# Autodesk Inventor assembly: Omni_Section
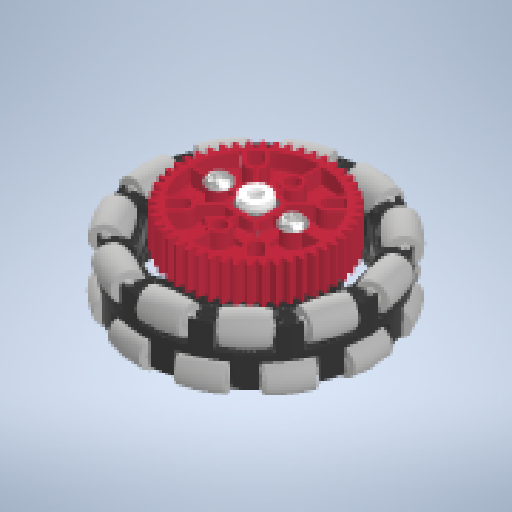
[picture p0: Inventor's stored thumbnail of the model, 512x512]
Saved by Autodesk Inventor 2025.2 (Build 292293000, 293)
## iProperties
Created: 2024-12-08
Part Number: Omni_Section
Document SubType Name: Assembly
Designer: Aditya Koduri
Author: Aditya Koduri
## Documents named in this file (13)
- C:\Users\joshi\Desktop\3388K CAD\Omni_Section.iam
- C:\Users\joshi\Desktop\3388K CAD\VEX Main\Structure\Hardware\Screw Steel - Hex\SScrew Hex Smooth 1.250.ipt
- C:\Users\joshi\Desktop\3388K CAD\VEX Main\Motion\Gears\HS Gear\HS 48T Gear, No Insert.iam
- C:\Users\joshi\Desktop\3388K CAD\VEX Main\Structure\Hardware\Nut Thin Nylock.ipt
- C:\Users\joshi\Desktop\3388K CAD\VEX Main\Motion\Wheels\Omni Wheel\3.25 Omni, No Insert.iam
- C:\Users\joshi\Desktop\3388K CAD\VEX Main\Motion\Insert Circle.ipt
- C:\Users\joshi\Desktop\3388K CAD\VEX Main\Motion\Spacers\Washer Teflon\TWasher .375 OD x .03125.ipt
- C:\Users\joshi\Desktop\3388K CAD\VEX Main\Motion\Spacers\Spacer Nylon .313 OD\NSpacer .313 OD x .250.ipt
- C:\Users\mzart\Downloads\VEX-CAD-Inventor-main\VEX-CAD-Inventor-main\Structure\Hardware\Screw Steel - Hex.ipt
- C:\Users\mzart\Downloads\VEX-CAD-Inventor-main\VEX-CAD-Inventor-main\Motion\Gears\HS Gear.iam
- C:\Users\mzart\Downloads\VEX-CAD-Inventor-main\VEX-CAD-Inventor-main\Motion\Wheels\Omni Wheel.iam
- C:\Users\mzart\Downloads\VEX-CAD-Inventor-main\VEX-CAD-Inventor-main\Motion\Spacers\Washer Teflon.ipt
- C:\Users\mzart\Downloads\VEX-CAD-Inventor-main\VEX-CAD-Inventor-main\Motion\Spacers\Spacer Nylon .313 OD.ipt
## Components (13 placed, 7 different names)
1. SScrew Hex Smooth 1.250:1
2. HS 48T Gear, No Insert:1 [sub-assembly] — Insert:10
3. Nut Thin Nylock:1
4. 3.25 Omni, No Insert:1 [sub-assembly] — Insert:11
5. SScrew Hex Smooth 1.250:2
6. Nut Thin Nylock:2
7. Insert Circle:1 — Insert:10, Insert:17
8. Insert Circle:2 — Insert:11, Insert:20
9. TWasher .375 OD x .03125:1 — Insert:18
10. TWasher .375 OD x .03125:2 — Insert:17, Insert:18
11. NSpacer .313 OD x .250:2 — Insert:19, Insert:20
12. TWasher .375 OD x .03125:3 — Insert:19, Insert:21
13. TWasher .375 OD x .03125:4 — Insert:21
## Relationships (13: Insert 13)
- [Insert]: HS 48T Gear, No Insert:1 ↔ 3.25 Omni, No Insert:1
- [Insert]: HS 48T Gear, No Insert:1 ↔ 3.25 Omni, No Insert:1
- [Insert]: SScrew Hex Smooth 1.250:1 ↔ HS 48T Gear, No Insert:1
- [Insert]: HS 48T Gear, No Insert:1 ↔ SScrew Hex Smooth 1.250:2
- [Insert]: Nut Thin Nylock:1 ↔ 3.25 Omni, No Insert:1
- [Insert]: 3.25 Omni, No Insert:1 ↔ Nut Thin Nylock:2
- Insert:10: HS 48T Gear, No Insert:1 ↔ Insert Circle:1
- Insert:11: 3.25 Omni, No Insert:1 ↔ Insert Circle:2
- Insert:17: Insert Circle:1 ↔ TWasher .375 OD x .03125:2
- Insert:18: TWasher .375 OD x .03125:1 ↔ TWasher .375 OD x .03125:2
- Insert:19: NSpacer .313 OD x .250:2 ↔ TWasher .375 OD x .03125:3
- Insert:20: Insert Circle:2 ↔ NSpacer .313 OD x .250:2
- Insert:21: TWasher .375 OD x .03125:3 ↔ TWasher .375 OD x .03125:4
